# Autodesk Inventor assembly: OBG-Elektronik
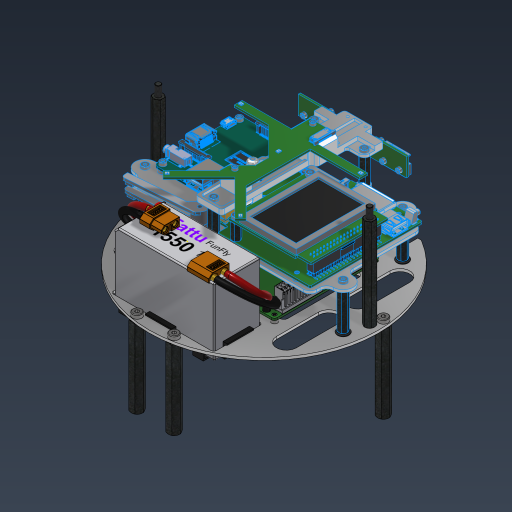
[picture p0: Inventor's stored thumbnail of the model, 512x512]
Saved by Autodesk Inventor 2023.1 (Build 271208000, 208)
## iProperties
Part Number: OBG-Elektronik
Material: Generisch
Document SubType Name: Assembly
Designer: rYan
Mass: 775.157 g
Surface Area: 2298.1 cm^2
Volume: 307.983 cm^3
Density: 2.51689 g/cm^3
Author: rYan
## Documents named in this file (14)
- D:\TIGERsGIT\Hardware\mechanik\2024\Inventor\Robot\Electronics\OBG-Elektronik.iam
- D:\TIGERsGIT\Hardware\mechanik\2024\Inventor\Robot\Electronics\Mittelplatte.ipt
- D:\TIGERsGIT\Hardware\mechanik\2024\Inventor\Inhaltscenter\de-DE\DIN 7984\DIN 7984 - M4 x 6.ipt
- D:\TIGERsGIT\Hardware\mechanik\2024\Inventor\Robot\Electronics\MG-Powerboard.iam
- D:\TIGERsGIT\Hardware\mechanik\2019\Inventor\Kaufteile\Abstandsbolzen Typ B.ipt
- D:\TIGERsGIT\Hardware\mechanik\2024\Inventor\Robot\Electronics\UBG-Compute Layer.iam
- D:\TIGERsGIT\Hardware\mechanik\2024\Inventor\Purchased Parts\Abstandsbolzen Typ B M4 70mm.ipt
- D:\TIGERsGIT\Hardware\mechanik\2024\Inventor\Robot\Electronics\Akkuhalter.ipt
- D:\TIGERsGIT\Hardware\mechanik\2024\Inventor\Purchased Parts\Gummitülle 3mm.ipt
- D:\TIGERsGIT\Hardware\mechanik\2024\Inventor\Inhaltscenter\de-DE\ISO 4762(2)\ISO 4762 - M2 x 6ISO.ipt
- D:\TIGERsGIT\Hardware\mechanik\2024\Inventor\Inhaltscenter\de-DE\ISO 10642(1)\ISO 10642 - M3 x  8.ipt
- D:\TIGERsGIT\Hardware\mechanik\2024\Inventor\Purchased Parts\MG-Akku 6S1P Tattu Funfly 1550mAh.iam
- D:\TIGERsGIT\Hardware\mechanik\2024\Inventor\Purchased Parts\Abstandsbolzen Typ A M4 60mm SW8.ipt
- D:\TIGERsGIT\Hardware\mechanik\2024\Inventor\Purchased Parts\Abstandsbolzen Typ A.ipt
## Components (29 placed, 11 different names)
1. Mittelplatte:1 — Einfügen:7, Einfügen:8, Fluchtend:1, Fluchtend:2, Fluchtend:3, Passend:19, Einfügen:34, Einfügen:36, Einfügen:42, Einfügen:43, Einfügen:44, Einfügen:45, Einfügen:55, Passend:25, Einfügen:56, Einfügen:57, Einfügen:58, Einfügen:59, Einfügen:64, Einfügen:65, Einfügen:66, Einfügen:67, Passend:28, Passend:29, Passend:30, Passend:36, Einfügen:75, Einfügen:76, Einfügen:77, Einfügen:78
2. DIN 7984 M4 x 6:1 — Einfügen:7
3. DIN 7984 M4 x 6:2 — Einfügen:8
4. MG-Powerboard:1 [sub-assembly] — Einfügen:55, Passend:25
5. UBG-Compute Layer:1 [sub-assembly] — Passend:19, Einfügen:50
6. DIN 7984 M4 x 6:4 — Einfügen:34
7. DIN 7984 M4 x 6:6 — Einfügen:36
8. Abstandsbolzen Typ B M4 70mm:5 — Einfügen:42
9. Abstandsbolzen Typ B M4 70mm:6 — Einfügen:43
10. DIN 7984 M4 x 6:7 — Einfügen:44
11. DIN 7984 M4 x 6:8 — Einfügen:45
12. Akkuhalter:1 — Passend:28, Passend:29, Passend:30, Passend:35, Passend:37
13. Gummitülle 3mm:1 — Einfügen:64, Einfügen:73
14. Gummitülle 3mm:2 — Einfügen:50, Einfügen:65, Einfügen:74
15. Gummitülle 3mm:3 — Einfügen:66, Einfügen:72
16. Gummitülle 3mm:4 — Einfügen:67, Einfügen:71
17. ISO 4762 M2 x 6:1 — Einfügen:58
18. ISO 4762 M2 x 6:2 — Einfügen:59
19. ISO 4762 M2 x 6:3 — Einfügen:57
20. ISO 4762 M2 x 6:4 — Einfügen:56
21. ISO 10642 M3 x  8:1 — Einfügen:73
22. ISO 10642 M3 x  8:2 — Einfügen:74
23. ISO 10642 M3 x  8:3 — Einfügen:72
24. ISO 10642 M3 x  8:4 — Einfügen:71
25. MG-Akku 6S1P Tattu Funfly 1550mAh:1 [sub-assembly] — Passend:35, Passend:36, Passend:37
26. Abstandsbolzen Typ A M4 60mm SW8:1 — Einfügen:75
27. Abstandsbolzen Typ A M4 60mm SW8:2 — Einfügen:78
28. Abstandsbolzen Typ A M4 60mm SW8:3 — Einfügen:77
29. Abstandsbolzen Typ A M4 60mm SW8:4 — Einfügen:76
## Relationships (37: Insert 26, Mate 8, Flush 3)
- Einfügen:7 [Insert]: Mittelplatte:1 ↔ DIN 7984 M4 x 6:1
- Einfügen:8 [Insert]: Mittelplatte:1 ↔ DIN 7984 M4 x 6:2
- Fluchtend:1 [Flush]: Mittelplatte:1
- Fluchtend:2 [Flush]: Mittelplatte:1
- Fluchtend:3 [Flush]: Mittelplatte:1
- Passend:19 [Mate]: Mittelplatte:1 ↔ UBG-Compute Layer:1
- Einfügen:34 [Insert]: Mittelplatte:1 ↔ DIN 7984 M4 x 6:4
- Einfügen:36 [Insert]: Mittelplatte:1 ↔ DIN 7984 M4 x 6:6
- Einfügen:42 [Insert]: Mittelplatte:1 ↔ Abstandsbolzen Typ B M4 70mm:5
- Einfügen:43 [Insert]: Mittelplatte:1 ↔ Abstandsbolzen Typ B M4 70mm:6
- Einfügen:44 [Insert]: Mittelplatte:1 ↔ DIN 7984 M4 x 6:7
- Einfügen:45 [Insert]: Mittelplatte:1 ↔ DIN 7984 M4 x 6:8
- Einfügen:50 [Insert]: UBG-Compute Layer:1 ↔ Gummitülle 3mm:2
- Einfügen:55 [Insert]: Mittelplatte:1 ↔ MG-Powerboard:1
- Passend:25 [Mate]: Mittelplatte:1 ↔ MG-Powerboard:1
- Einfügen:56 [Insert]: Mittelplatte:1 ↔ ISO 4762 M2 x 6:4
- Einfügen:57 [Insert]: Mittelplatte:1 ↔ ISO 4762 M2 x 6:3
- Einfügen:58 [Insert]: Mittelplatte:1 ↔ ISO 4762 M2 x 6:1
- Einfügen:59 [Insert]: Mittelplatte:1 ↔ ISO 4762 M2 x 6:2
- Einfügen:64 [Insert]: Mittelplatte:1 ↔ Gummitülle 3mm:1
- Einfügen:65 [Insert]: Mittelplatte:1 ↔ Gummitülle 3mm:2
- Einfügen:66 [Insert]: Mittelplatte:1 ↔ Gummitülle 3mm:3
- Einfügen:67 [Insert]: Mittelplatte:1 ↔ Gummitülle 3mm:4
- Passend:28 [Mate] (0.1 mm): Mittelplatte:1 ↔ Akkuhalter:1
- Passend:29 [Mate] (0.1 mm): Mittelplatte:1 ↔ Akkuhalter:1
- Passend:30 [Mate]: Mittelplatte:1 ↔ Akkuhalter:1
- Einfügen:71 [Insert] (-0.5 mm): Gummitülle 3mm:4 ↔ ISO 10642 M3 x  8:4
- Einfügen:72 [Insert] (-0.5 mm): Gummitülle 3mm:3 ↔ ISO 10642 M3 x  8:3
- Einfügen:73 [Insert] (-0.5 mm): Gummitülle 3mm:1 ↔ ISO 10642 M3 x  8:1
- Einfügen:74 [Insert] (-0.5 mm): Gummitülle 3mm:2 ↔ ISO 10642 M3 x  8:2
- Passend:35 [Mate]: Akkuhalter:1 ↔ MG-Akku 6S1P Tattu Funfly 1550mAh:1
- Passend:36 [Mate]: Mittelplatte:1 ↔ MG-Akku 6S1P Tattu Funfly 1550mAh:1
- Passend:37 [Mate]: Akkuhalter:1 ↔ MG-Akku 6S1P Tattu Funfly 1550mAh:1
- Einfügen:75 [Insert]: Mittelplatte:1 ↔ Abstandsbolzen Typ A M4 60mm SW8:1
- Einfügen:76 [Insert]: Mittelplatte:1 ↔ Abstandsbolzen Typ A M4 60mm SW8:4
- Einfügen:77 [Insert]: Mittelplatte:1 ↔ Abstandsbolzen Typ A M4 60mm SW8:3
- Einfügen:78 [Insert]: Mittelplatte:1 ↔ Abstandsbolzen Typ A M4 60mm SW8:2
